# Autodesk Inventor assembly: PotentiometerAssembly
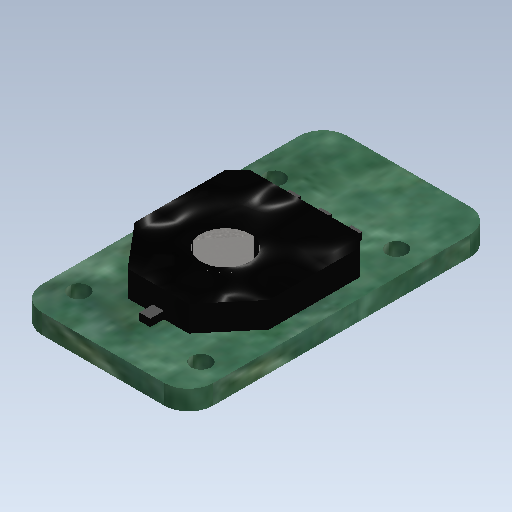
[picture p0: Inventor's stored thumbnail of the model, 512x512]
Saved by Autodesk Inventor 2020.2 (Build 242310000, 310)
## iProperties
Created: 2020-01-18
Part Number: PotentiometerAssembly
Document SubType Name: Assembly
Designer: sami_
Author: sami_
## Documents named in this file (4)
- C:\Users\PROXS\Desktop\Curved Hand 100319 Ver - Shaft inc22\Curved Hand 100319 Ver - Shaft inc\Workgroups\NotInProject\THUMB\Assembly\PotentiometerAssembly.iam
- C:\Users\PROXS\Desktop\Curved Hand 100319 Ver - Shaft inc22\Curved Hand 100319 Ver - Shaft inc\Workgroups\NotInProject\THUMB\Assembly\potentiometerbody.ipt
- C:\Users\PROXS\Desktop\Curved Hand 100319 Ver - Shaft inc22\Curved Hand 100319 Ver - Shaft inc\Workgroups\NotInProject\THUMB\Assembly\potentiometerspinny.ipt
- C:\Users\PROXS\Desktop\Curved Hand 100319 Ver - Shaft inc22\Curved Hand 100319 Ver - Shaft inc\Workgroups\NotInProject\THUMB\Assembly\potentiometerpcb.ipt
## Components (3 placed, 3 different names)
1. potentiometerbody:1 — Rotational:1, Rigid:1
2. potentiometerspinny:1 — Rotational:1
3. potentiometerpcb:1 — Rigid:1
## Relationships (2: RevoluteJoint 1, WeldJoint 1)
- Rotational:1 [RevoluteJoint] (0.02 mm): potentiometerbody:1 ↔ potentiometerspinny:1
- Rigid:1 [WeldJoint]: potentiometerbody:1 ↔ potentiometerpcb:1
